# Autodesk Inventor assembly: Elastic Horizontal Roller
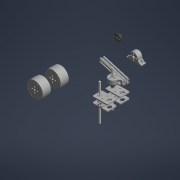
[picture p0: Inventor's stored thumbnail of the model, 180x180]
Saved by Autodesk Inventor 2022 (Build 260153000, 153)
## iProperties
Part Number: Elastic Horizontal Roller
Document SubType Name: Assembly
Designer: izack
Author: izack
## Documents named in this file (10)
- F:\CAD Modeling\GithubCAD\ComputerAidedDesign\2021-22\FTC\#12456 Big Red\Out Take\Elastic Horizontal Rollers\Elastic Horizontal Roller.iam
- F:\CAD Modeling\GithubCAD\ComputerAidedDesign\2021-22\FTC\#12456 Big Red\Out Take\Bearing Bushing.ipt
- F:\CAD Modeling\GithubCAD\ComputerAidedDesign\2021-22\FTC\#12456 Big Red\Out Take\Elastic Horizontal Rollers\15mm Extrusion - 420mm.ipt
- F:\CAD Modeling\GithubCAD\ComputerAidedDesign\2021-22\FTC\#12456 Big Red\Out Take\Elastic Horizontal Rollers\2in 5mm Hex Stealth Wheel.iam
- F:\CAD Modeling\GithubCAD\ComputerAidedDesign\2021-22\FTC\#12456 Big Red\Out Take\Elastic Horizontal Rollers\8mm x 12mm x 3.5mm Flanged Bearing.ipt
- F:\CAD Modeling\GithubCAD\ComputerAidedDesign\2021-22\FTC\#12456 Big Red\Out Take\Elastic Horizontal Rollers\5mm Hex to 8mm Round Bearing Insert - 20 Pack.ipt
- F:\CAD Modeling\GithubCAD\ComputerAidedDesign\2021-22\FTC\#12456 Big Red\Out Take\Elastic Horizontal Rollers\5mm x 100mm Hex Shaft - 4 Pack.ipt
- F:\CAD Modeling\GithubCAD\ComputerAidedDesign\2021-22\FTC\#12456 Big Red\Out Take\Elastic Horizontal Rollers\15mm Hex Hub.ipt
- F:\CAD Modeling\GithubCAD\ComputerAidedDesign\2021-22\FTC\#12456 Big Red\Out Take\Elastic Horizontal Rollers\15mm Extrusion - 100mm.ipt
- F:\CAD Modeling\GithubCAD\ComputerAidedDesign\2021-22\FTC\#12456 Big Red\Out Take\Elastic Horizontal Rollers\High Strength Hex Hub - 2 Pack.ipt
## Components (22 placed, 8 different names)
1. Bearing Bushing:1 — Mate:1, Flush:2, Mate:5, Mate:11, Flush:4, Flush:9
2. Bearing Bushing:2 — Mate:3, Flush:1, Mate:7, Mate:12, Flush:3, Flush:4, Flush:6
3. Bearing Bushing:3 — Mate:4, Mate:8, Mate:9, Flush:5, Flush:6, Flush:7
4. Bearing Bushing:4 — Mate:2, Mate:6, Mate:10, Flush:5, Flush:8
5. 15mm Extrusion - 70mm:1 — Mate:1, Mate:2, Mate:3, Mate:4, Flush:1, Flush:2, Flush:3, Flush:7, Flush:8, Flush:9
6. 2in 5mm Hex Stealth Wheel:1 [sub-assembly]
7. 2in 5mm Hex Stealth Wheel:2 [sub-assembly]
8. 8mm x 12mm x 3.5mm Flanged Bearing:1 — Mate:6, Mate:10, Mate:13, Mate:19
9. 8mm x 12mm x 3.5mm Flanged Bearing:2 — Mate:7, Mate:12, Mate:16, Mate:17
10. 8mm x 12mm x 3.5mm Flanged Bearing:3 — Mate:8, Mate:9, Mate:15, Mate:18
11. 8mm x 12mm x 3.5mm Flanged Bearing:4 — Mate:5, Mate:11, Mate:14, Mate:20
12. 5mm Hex to 8mm Round Bearing Insert - 20 Pack:1 — Mate:13, Mate:19, Mate:23, Mate:24, Mate:29
13. 5mm Hex to 8mm Round Bearing Insert - 20 Pack:2 — Mate:14, Mate:20, Mate:21, Mate:22
14. 5mm Hex to 8mm Round Bearing Insert - 20 Pack:3 — Mate:16, Mate:17
15. 5mm Hex to 8mm Round Bearing Insert - 20 Pack:4 — Mate:15, Mate:18
16. 5mm x 100mm Hex Shaft - 4 Pack:1 — Mate:21, Mate:22
17. 5mm x 100mm Hex Shaft - 4 Pack:2 — Mate:23, Mate:24, Mate:30, Mate:31
18. 15mm Hex Hub:1
19. 15mm Hex Hub:2 — Mate:25, Flush:10, Flush:11, Mate:26, Mate:27, Mate:28
20. 15mm Extrusion - 70mm:2 — Mate:25, Flush:10, Flush:11
21. High Strength Hex Hub - 2 Pack:1 — Mate:26, Mate:27, Mate:28, Mate:29, Mate:30, Mate:31
22. High Strength Hex Hub - 2 Pack:2
## Relationships (42: Mate 31, Flush 11)
- Mate:1: Bearing Bushing:1 ↔ 15mm Extrusion - 70mm:1
- Mate:2: Bearing Bushing:4 ↔ 15mm Extrusion - 70mm:1
- Mate:3: Bearing Bushing:2 ↔ 15mm Extrusion - 70mm:1
- Mate:4: Bearing Bushing:3 ↔ 15mm Extrusion - 70mm:1
- Flush:1: Bearing Bushing:2 ↔ 15mm Extrusion - 70mm:1
- Flush:2: Bearing Bushing:1 ↔ 15mm Extrusion - 70mm:1
- Mate:5: Bearing Bushing:1 ↔ 8mm x 12mm x 3.5mm Flanged Bearing:4
- Mate:6: Bearing Bushing:4 ↔ 8mm x 12mm x 3.5mm Flanged Bearing:1
- Mate:7: Bearing Bushing:2 ↔ 8mm x 12mm x 3.5mm Flanged Bearing:2
- Mate:8: Bearing Bushing:3 ↔ 8mm x 12mm x 3.5mm Flanged Bearing:3
- Mate:9: Bearing Bushing:3 ↔ 8mm x 12mm x 3.5mm Flanged Bearing:3
- Mate:10: Bearing Bushing:4 ↔ 8mm x 12mm x 3.5mm Flanged Bearing:1
- Mate:11: Bearing Bushing:1 ↔ 8mm x 12mm x 3.5mm Flanged Bearing:4
- Mate:12: Bearing Bushing:2 ↔ 8mm x 12mm x 3.5mm Flanged Bearing:2
- Mate:13: 8mm x 12mm x 3.5mm Flanged Bearing:1 ↔ 5mm Hex to 8mm Round Bearing Insert - 20 Pack:1
- Mate:14: 8mm x 12mm x 3.5mm Flanged Bearing:4 ↔ 5mm Hex to 8mm Round Bearing Insert - 20 Pack:2
- Mate:15: 8mm x 12mm x 3.5mm Flanged Bearing:3 ↔ 5mm Hex to 8mm Round Bearing Insert - 20 Pack:4
- Mate:16: 8mm x 12mm x 3.5mm Flanged Bearing:2 ↔ 5mm Hex to 8mm Round Bearing Insert - 20 Pack:3
- Mate:17: 8mm x 12mm x 3.5mm Flanged Bearing:2 ↔ 5mm Hex to 8mm Round Bearing Insert - 20 Pack:3
- Mate:18: 8mm x 12mm x 3.5mm Flanged Bearing:3 ↔ 5mm Hex to 8mm Round Bearing Insert - 20 Pack:4
- Mate:19: 8mm x 12mm x 3.5mm Flanged Bearing:1 ↔ 5mm Hex to 8mm Round Bearing Insert - 20 Pack:1
- Mate:20: 8mm x 12mm x 3.5mm Flanged Bearing:4 ↔ 5mm Hex to 8mm Round Bearing Insert - 20 Pack:2
- Flush:3 (-16 mm): Bearing Bushing:2 ↔ 15mm Extrusion - 70mm:1
- Flush:4: Bearing Bushing:1 ↔ Bearing Bushing:2
- Flush:5: Bearing Bushing:3 ↔ Bearing Bushing:4
- Flush:6: Bearing Bushing:2 ↔ Bearing Bushing:3
- Flush:7: Bearing Bushing:3 ↔ 15mm Extrusion - 70mm:1
- Flush:8: Bearing Bushing:4 ↔ 15mm Extrusion - 70mm:1
- Flush:9: Bearing Bushing:1 ↔ 15mm Extrusion - 70mm:1
- Mate:21: 5mm Hex to 8mm Round Bearing Insert - 20 Pack:2 ↔ 5mm x 100mm Hex Shaft - 4 Pack:1
- Mate:22: 5mm Hex to 8mm Round Bearing Insert - 20 Pack:2 ↔ 5mm x 100mm Hex Shaft - 4 Pack:1
- Mate:23: 5mm Hex to 8mm Round Bearing Insert - 20 Pack:1 ↔ 5mm x 100mm Hex Shaft - 4 Pack:2
- Mate:24: 5mm Hex to 8mm Round Bearing Insert - 20 Pack:1 ↔ 5mm x 100mm Hex Shaft - 4 Pack:2
- Mate:25: 15mm Hex Hub:2 ↔ 15mm Extrusion - 70mm:2
- Flush:10: 15mm Hex Hub:2 ↔ 15mm Extrusion - 70mm:2
- Flush:11: 15mm Hex Hub:2 ↔ 15mm Extrusion - 70mm:2
- Mate:26: 15mm Hex Hub:2 ↔ High Strength Hex Hub - 2 Pack:1
- Mate:27: 15mm Hex Hub:2 ↔ High Strength Hex Hub - 2 Pack:1
- Mate:28: 15mm Hex Hub:2 ↔ High Strength Hex Hub - 2 Pack:1
- Mate:29: 5mm Hex to 8mm Round Bearing Insert - 20 Pack:1 ↔ High Strength Hex Hub - 2 Pack:1
- Mate:30: 5mm x 100mm Hex Shaft - 4 Pack:2 ↔ High Strength Hex Hub - 2 Pack:1
- Mate:31: 5mm x 100mm Hex Shaft - 4 Pack:2 ↔ High Strength Hex Hub - 2 Pack:1
